# Autodesk Inventor assembly: v4assembly
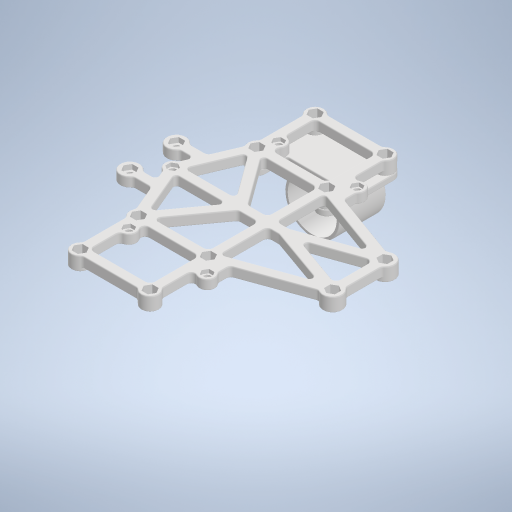
[picture p0: Inventor's stored thumbnail of the model, 512x512]
Saved by Autodesk Inventor 2024.2 (Build 282272000, 272)
## iProperties
Created: 2024-02-10
Part Number: v4assembly
Document SubType Name: Assembly
Designer: Eric
Author: Eric
## Documents named in this file (3)
- C:\Users\Eric\Desktop\scioly-robot-tour\Hardware\ipt\v4\v4assembly.iam
- C:\Users\Eric\Desktop\scioly-robot-tour\Hardware\ipt\v4\v4motormount.ipt
- C:\Users\Eric\Desktop\scioly-robot-tour\Hardware\ipt\v4\v4chassisv2.ipt
## Components (2 placed, 2 different names)
1. v4chassisv2:1 — Mate:1, Tangent:1, Tangent:2
2. v4motormount:2 — Mate:1, Tangent:1, Tangent:2
## Relationships (3: Tangent 2, Mate 1)
- Mate:1: v4chassisv2:1 ↔ v4motormount:2
- Tangent:1: v4chassisv2:1 ↔ v4motormount:2
- Tangent:2: v4chassisv2:1 ↔ v4motormount:2
